# Autodesk Inventor assembly: RSF-11B
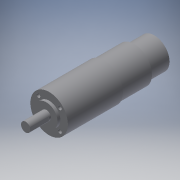
[picture p0: Inventor's stored thumbnail of the model, 180x180]
Saved by Autodesk Inventor 2016 (Build 200138000, 138)
## iProperties
Created: 2016-06-23
Part Number: RSF-11B
Material: 一般
Document SubType Name: Assembly
Designer: 宏太
Author: 宏太
## Documents named in this file (5)
- C:\Users\宏太\Documents\Inventor\Content Center Files\Tomoto2016\RSF-11B\RSF-11B.iam
- C:\Users\宏太\Documents\Inventor\Content Center Files\Tomoto2016\RSF-11B\encorder.ipt
- C:\Users\宏太\Documents\Inventor\Content Center Files\Tomoto2016\RSF-11B\HarmonicDrive1.ipt
- C:\Users\宏太\Documents\Inventor\Content Center Files\Tomoto2016\RSF-11B\motor.ipt
- C:\Users\宏太\Documents\Inventor\Content Center Files\Tomoto2016\RSF-11B\shaft.ipt
## Components (4 placed, 4 different names)
1. encorder:1 — 挿入:1
2. HarmonicDrive1:1 — 挿入:2, 挿入:3
3. motor:1 — 挿入:1, 挿入:2
4. shaft:1 — 挿入:3
## Relationships (3: Insert 3)
- 挿入:1 [Insert]: encorder:1 ↔ motor:1
- 挿入:2 [Insert]: HarmonicDrive1:1 ↔ motor:1
- 挿入:3 [Insert]: HarmonicDrive1:1 ↔ shaft:1
